# Autodesk Inventor assembly: Individual Hook
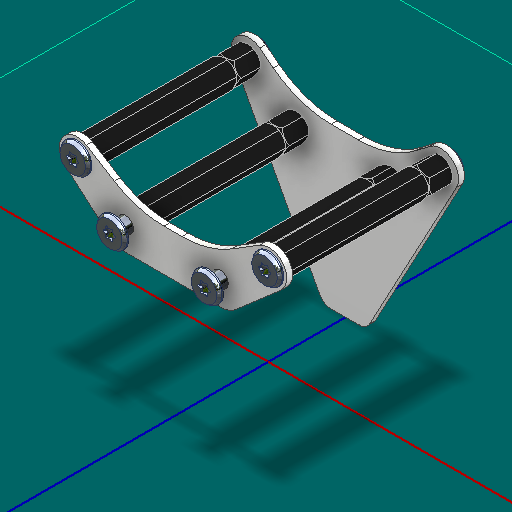
[picture p0: Inventor's stored thumbnail of the model, 512x512]
Saved by Autodesk Inventor 2025 (Build 290162000, 162)
## iProperties
Created: 2024-10-22
Part Number: Individual Hook
Document SubType Name: Assembly
Designer: averey
Author: averey
## Documents named in this file (8)
- C:\Users\avere\VEX\High Stakes\CAD\V2\Hook\Individual Hook.iam
- C:\Users\avere\VEX\High Stakes\CAD\V2\Hook\Custom Parts\Hook Gusset.ipt
- C:\Users\avere\VEX\High Stakes\CAD\ROBOPROS-CAD-Inventor\Structure\Standoff\Standoff .25.ipt
- C:\Users\avere\VEX\High Stakes\CAD\ROBOPROS-CAD-Inventor\Structure\Standoff.ipt
- C:\Users\avere\VEX\High Stakes\CAD\ROBOPROS-CAD-Inventor\Structure\Hardware\Screw Shoulder Robosource\SScrew Shoulder Smooth .500 x .04.ipt
- C:\Users\avere\VEX\High Stakes\CAD\ROBOPROS-CAD-Inventor\Structure\Hardware\Screw Shoulder Robosource.ipt
- C:\Users\avere\VEX\High Stakes\CAD\ROBOPROS-CAD-Inventor\Structure\Standoff\Standoff 1.50.ipt
- C:\Users\avere\VEX\High Stakes\CAD\V2\Hook\Custom Parts\Hook Gusset Brace.ipt
## Components (18 placed, 5 different names)
1. Hook Gusset:1 — Mate:3
2. Standoff .25:1
3. Standoff .25:2
4. SScrew Shoulder Smooth .500 x .04:1
5. SScrew Shoulder Smooth .500 x .04:2
6. Standoff 1.50:3
7. Standoff 1.50:4
8. Standoff .25:5
9. Standoff 1.50:6
10. Standoff .25:7
11. Standoff 1.50:8
12. Hook Gusset Brace:1 — Flush:1, Mate:4
13. SScrew Shoulder Smooth .500 x .04:3
14. SScrew Shoulder Smooth .500 x .04:4
15. SScrew Shoulder Smooth .500 x .04:5
16. SScrew Shoulder Smooth .500 x .04:6
17. SScrew Shoulder Smooth .500 x .04:7
18. SScrew Shoulder Smooth .500 x .04:8
## Relationships (22: Insert 17, Mate 4, Flush 1)
- [Insert]: Hook Gusset:1 ↔ Standoff .25:1
- [Insert]: Hook Gusset:1 ↔ SScrew Shoulder Smooth .500 x .04:2
- [Insert]: Hook Gusset:1 ↔ SScrew Shoulder Smooth .500 x .04:1
- [Mate]: Standoff .25:2 ↔ SScrew Shoulder Smooth .500 x .04:2
- [Insert]: Hook Gusset:1 ↔ Standoff .25:5
- [Insert]: Standoff 1.50:3 ↔ Standoff .25:5
- [Insert]: Hook Gusset:1 ↔ Standoff .25:2
- [Insert]: Standoff .25:2 ↔ Standoff 1.50:6
- [Insert]: Standoff .25:1 ↔ Standoff 1.50:4
- [Insert]: Standoff .25:7 ↔ Standoff 1.50:8
- [Insert]: Hook Gusset:1 ↔ Standoff .25:7
- [Insert]: Standoff 1.50:8 ↔ Hook Gusset Brace:1
- [Mate]: Standoff 1.50:4 ↔ Hook Gusset Brace:1
- [Insert]: Hook Gusset:1 ↔ SScrew Shoulder Smooth .500 x .04:3
- [Insert]: Hook Gusset:1 ↔ SScrew Shoulder Smooth .500 x .04:4
- [Insert]: Hook Gusset Brace:1 ↔ SScrew Shoulder Smooth .500 x .04:6
- [Insert]: Hook Gusset Brace:1 ↔ SScrew Shoulder Smooth .500 x .04:5
- [Insert] (3.175 mm): Hook Gusset Brace:1 ↔ SScrew Shoulder Smooth .500 x .04:7
- [Insert] (3.175 mm): Hook Gusset Brace:1 ↔ SScrew Shoulder Smooth .500 x .04:8
- Mate:3 (-22.225 mm): Hook Gusset:1
- Flush:1: Hook Gusset Brace:1
- Mate:4 (2.402 mm): Hook Gusset Brace:1
## Named parameters: d19_d5 = 0 mm, d20_d6 = 0 mm, d21_d7 = 0 mm, d83_d82 = 0 mm
